# Autodesk Inventor assembly: Frame
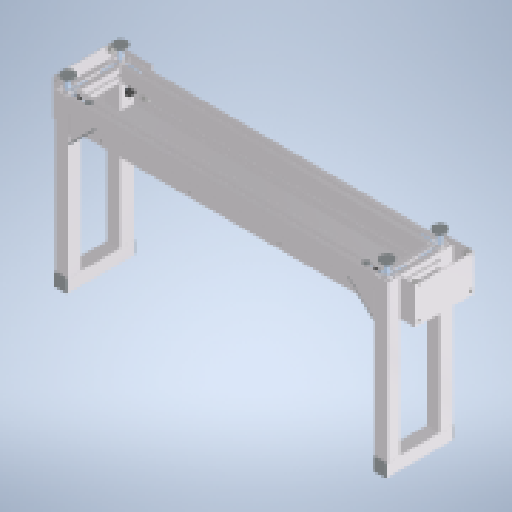
[picture p0: Inventor's stored thumbnail of the model, 512x512]
Saved by Autodesk Inventor 2025 (Build 290162010, 162A)
## iProperties
Created: 2025-01-18
Part Number: Frame
Document SubType Name: Assembly
Designer: Admin
Author: Admin
## Documents named in this file (34)
- C:\Users\Admin\GIT\HDVKBM\CAD\Krandemonstrator\Frame.iam
- C:\Users\Admin\GIT\HDVKBM\CAD\Krandemonstrator\item_61193_profil-x-8-40x40-2no180-_930_high\item_61193_profil-x-8-40x40-2no180-_930_high.ipt
- C:\Users\Admin\GIT\HDVKBM\CAD\Krandemonstrator\item_49291_profil-x-8-40x40-leicht-_120_high\item_49291_profil-x-8-40x40-leicht-_120_high.ipt
- C:\Users\Admin\GIT\HDVKBM\CAD\Krandemonstrator\item_49288_profil-x-8-40x40-4no-lei_200_high\item_49288_profil-x-8-40x40-4no-lei_200_high.ipt
- C:\Users\Admin\GIT\HDVKBM\CAD\Krandemonstrator\item_49288_profil-x-8-40x40-4no-lei_475_high\item_49288_profil-x-8-40x40-4no-lei_475_high.ipt
- C:\Users\Admin\GIT\HDVKBM\CAD\Krandemonstrator\item_67284_automatik-verbindungssat__high\item_67284_automatik-verbindungssat__high.ipt
- C:\Users\Admin\GIT\HDVKBM\CAD\Krandemonstrator\item_63697_stellfuss-d40-m8x60-grau_35_0_high\item_63697_stellfuss-d40-m8x60-grau_35_0_high.ipt
- C:\Users\Admin\GIT\HDVKBM\CAD\Krandemonstrator\item_62716_abdeckkappe-8-40x40-grau__high\item_62716_abdeckkappe-8-40x40-grau__high.ipt
- C:\Users\Admin\GIT\HDVKBM\CAD\Krandemonstrator\item_48996_automatik-verbindungssat__high\item_48996_automatik-verbindungssat__high.ipt
- C:\Users\Admin\GIT\HDVKBM\CAD\Krandemonstrator\item_41123_winkel-8-80x80-zn-weissa__high\item_41123_winkel-8-80x80-zn-weissa__high.ipt
- C:\Users\Admin\GIT\HDVKBM\CAD\Krandemonstrator\item_2618_nutenstein-8-st-m8-verzi__high\item_2618_nutenstein-8-st-m8-verzi__high.ipt
- C:\Users\Admin\Documents\Inventor\Content Center Files\R2025\de-DE\AS 1420\AS 1420 - 1973 - M8 x 16.ipt
- C:\Users\Admin\GIT\HDVKBM\CAD\Krandemonstrator\item_62758_winkel-abdeckkappe-8-80x__high\item_62758_winkel-abdeckkappe-8-80x__high.ipt
- C:\Users\Admin\GIT\HDVKBM\CAD\Krandemonstrator\item_43452_stellfuss-d30-m6x45-schw_20_0_high\item_43452_stellfuss-d30-m6x45-schw_20_0_high.ipt
- C:\Users\Admin\GIT\HDVKBM\CAD\Krandemonstrator\item_2623_nutenstein-8-st-m6-verzi__high\item_2623_nutenstein-8-st-m6-verzi__high.ipt
- C:\Users\Admin\GIT\HDVKBM\CAD\Krandemonstrator\item_42005_nutenstein-8-st-m5-verzi__high\item_42005_nutenstein-8-st-m5-verzi__high.ipt
- C:\Users\Admin\GIT\HDVKBM\CAD\Krandemonstrator\item_67777_winkel-5-20-weissalumini__high\item_67777_winkel-5-20-weissalumini__high.ipt
- C:\Users\Admin\GIT\HDVKBM\CAD\Krandemonstrator\item_68092_befestigungssatz-5-2-4mm_2_high\item_68092_befestigungssatz-5-2-4mm_2_high.ipt
- C:\Users\Admin\Documents\Inventor\Content Center Files\R2025\de-DE\DIN 7991(2)\DIN 7991 - M5x12.ipt
- C:\Users\Admin\GIT\HDVKBM\CAD\Krandemonstrator\item_47308_blech-al-2mm-naturfarben_1100_180_high\item_47308_blech-al-2mm-naturfarben_1100_180_high.ipt
- C:\Users\Admin\Documents\Inventor\Content Center Files\R2025\de-DE\DIN 7991(2)\DIN 7991 - M5x16.ipt
- C:\Users\Admin\Documents\Inventor\Content Center Files\R2025\de-DE\DIN 7991(2)\DIN 7991 - M4x8.ipt
- C:\Users\Admin\GIT\HDVKBM\CAD\Krandemonstrator\item_37006_nutenstein-5-st-m4-verzi__high\item_37006_nutenstein-5-st-m4-verzi__high.ipt
- C:\Users\Admin\GIT\HDVKBM\CAD\Krandemonstrator\item_47308_blech-al-2mm-naturfarben_110_1100_high\item_47308_blech-al-2mm-naturfarben_110_1100_high.ipt
- C:\Users\Admin\GIT\HDVKBM\CAD\Krandemonstrator\item_37003_profil-5-20x20-natur-370_1096_high\item_37003_profil-5-20x20-natur-370_1096_high.ipt
- C:\Users\Admin\GIT\HDVKBM\CAD\Krandemonstrator\item_43774_profil-5-20x20-1n-natur-_1096_high\item_43774_profil-5-20x20-1n-natur-_1096_high.ipt
- C:\Users\Admin\GIT\HDVKBM\CAD\Krandemonstrator\item_47308_blech-al-2mm-naturfarben_178_110_high\item_47308_blech-al-2mm-naturfarben_178_110_high.ipt
- C:\Users\Admin\GIT\HDVKBM\CAD\Krandemonstrator\item_47308_blech-al-2mm-naturfarben_120_90_high\item_47308_blech-al-2mm-naturfarben_120_90_high.ipt
- C:\Users\Admin\Documents\Inventor\Content Center Files\R2025\de-DE\DIN 7991(1)\DIN 7991 - M5  x  10.ipt
- C:\Users\Admin\GIT\HDVKBM\CAD\Krandemonstrator\Frameblock.ipt
- C:\Users\Admin\GIT\HDVKBM\CAD\Krandemonstrator\item_47308_blech-al-2mm-naturfarben_120_90_high\item_47308_blech-al-2mm-naturfarben_120_90_highLH.ipt
- C:\Users\Admin\Documents\Inventor\Content Center Files\R2025\de-DE\DIN 7991(2)\DIN 7991 - M3x8.ipt
- C:\Users\Admin\Documents\Inventor\Content Center Files\R2025\de-DE\DIN 7991(2)\DIN 7991 - M4x20.ipt
- C:\Users\Admin\Documents\Inventor\Content Center Files\R2025\de-DE\DIN 7991(1)\DIN 7991 - M4  x  8.ipt
## Components (126 placed, 33 different names)
1. Frameblock:1 — Starr:73, Starr:84, Passend:24
2. Frameblock:2 — Starr:74, Starr:83, Passend:23
3. Frameblock:3 — Starr:75
4. Frameblock:4 — Starr:76, Passend:16, Starr:82
5. Frameblock:5 — Starr:78
6. Frameblock:6 — Starr:77, Starr:81, Passend:11
7. Frameblock:7 — Starr:79
8. Frameblock:8 — Starr:80
9. DIN 7991 M3x8:1 — Passend:9
10. DIN 7991 M3x8:2 — Passend:10
11. item_37006_nutenstein-5-st-m4-verzi__high:5 — Starr:81
12. item_37006_nutenstein-5-st-m4-verzi__high:6 — Starr:84
13. DIN 7991 M4x20:1 — Passend:11
14. DIN 7991 M3x8:3 — Passend:12
15. DIN 7991 M3x8:4 — Passend:13
16. DIN 7991 M3x8:5 — Passend:14
17. DIN 7991 M3x8:6 — Passend:15
18. DIN 7991 M4x20:2 — Passend:16
19. item_37006_nutenstein-5-st-m4-verzi__high:7 — Starr:82
20. item_37006_nutenstein-5-st-m4-verzi__high:8 — Starr:83
21. DIN 7991 M3x8:7 — Passend:17
22. DIN 7991 M3x8:8 — Passend:18
23. DIN 7991 M3x8:9 — Passend:19
24. DIN 7991 M3x8:10 — Passend:20
25. DIN 7991 M3x8:11 — Passend:21
26. DIN 7991 M3x8:12 — Passend:22
27. DIN 7991 M4x20:3 — Passend:23
28. DIN 7991 M4x20:4 — Passend:24
29. DIN 7991 - ersetzt durch DIN EN ISO 10642 M4  x  8:1 — Starr:85, Starr:91
30. DIN 7991 - ersetzt durch DIN EN ISO 10642 M4  x  8:2 — Starr:86, Starr:92
31. DIN 7991 - ersetzt durch DIN EN ISO 10642 M4  x  8:3 — Starr:87, Starr:89
32. DIN 7991 - ersetzt durch DIN EN ISO 10642 M4  x  8:4 — Starr:88, Starr:90
33. item_37006_nutenstein-5-st-m4-verzi__high:9 — Starr:91
34. item_37006_nutenstein-5-st-m4-verzi__high:10 — Starr:92
35. item_37006_nutenstein-5-st-m4-verzi__high:11 — Starr:90
36. item_37006_nutenstein-5-st-m4-verzi__high:12 — Starr:89
37. item_61193_profil-x-8-40x40-2no180-_930_high:1 — Starr:12, Starr:13, Starr:14
38. item_61193_profil-x-8-40x40-2no180-_930_high:2 — Starr:17, Starr:27, Planar:1, Planar:2, Starr:47, Starr:48, Planar:68, Verschiebbar:70
39. item_49291_profil-x-8-40x40-leicht-_120_high:1 — Starr:7, Starr:8, Starr:9
40. item_49291_profil-x-8-40x40-leicht-_120_high:2 — Starr:24, Starr:25, Starr:26
41. item_49288_profil-x-8-40x40-4no-lei_200_high:1 — Starr:18, Starr:19, Starr:21, Starr:23
42. item_49288_profil-x-8-40x40-4no-lei_200_high:2 — Starr:2, Starr:4, Starr:5, Starr:6
43. item_49288_profil-x-8-40x40-4no-lei_475_high:1 — Starr:20, Starr:21, Starr:28, Starr:41, Verschiebbar:6
44. item_49288_profil-x-8-40x40-4no-lei_475_high:2 — Starr:22, Starr:23, Starr:25, Starr:27, Starr:29, Verschiebbar:2, Verschiebbar:4
45. item_49288_profil-x-8-40x40-4no-lei_475_high:3 — Starr:3, Starr:4, Starr:11, Starr:17, Verschiebbar:1, Verschiebbar:3, Planar:71
46. item_49288_profil-x-8-40x40-4no-lei_475_high:4 — Starr:1, Starr:2, Starr:9, Starr:10, Starr:14, Starr:43, Verschiebbar:5
47. item_67284_automatik-verbindungssat__high:1 — Starr:1
48. item_67284_automatik-verbindungssat__high:2 — Starr:20
49. item_67284_automatik-verbindungssat__high:3 — Starr:3
50. item_67284_automatik-verbindungssat__high:11 — Starr:22
51. item_67284_automatik-verbindungssat__high:4 — Starr:24
52. item_67284_automatik-verbindungssat__high:12 — Starr:26
53. item_67284_automatik-verbindungssat__high:5 — Starr:12
54. item_67284_automatik-verbindungssat__high:6 — Starr:13
55. item_67284_automatik-verbindungssat__high:7 — Starr:8
56. item_67284_automatik-verbindungssat__high:8 — Starr:7
57. item_48996_automatik-verbindungssat__high:1 — Starr:47
58. item_48996_automatik-verbindungssat__high:2 — Starr:48
59. item_63697_stellfuss-d40-m8x60-grau_35_0_high:1 — Starr:10
60. item_63697_stellfuss-d40-m8x60-grau_35_0_high:2 — Starr:11
61. item_63697_stellfuss-d40-m8x60-grau_35_0_high:3 — Starr:28
62. item_63697_stellfuss-d40-m8x60-grau_35_0_high:4 — Starr:29
63. item_62716_abdeckkappe-8-40x40-grau__high:1 — Starr:5
64. item_62716_abdeckkappe-8-40x40-grau__high:2 — Starr:6
65. item_62716_abdeckkappe-8-40x40-grau__high:3 — Starr:18
66. item_62716_abdeckkappe-8-40x40-grau__high:4 — Starr:19
67. item_41123_winkel-8-80x80-zn-weissa__high:1 — Einfügen:3, Einfügen:4, Einfügen:7, Einfügen:8, Verschiebbar:2, Planar:2, Starr:38
68. item_41123_winkel-8-80x80-zn-weissa__high:2 — Einfügen:1, Einfügen:2, Einfügen:5, Einfügen:6, Verschiebbar:1, Planar:1, Starr:39
69. item_2618_nutenstein-8-st-m8-verzi__high:5 — Starr:37
70. item_2618_nutenstein-8-st-m8-verzi__high:3 — Starr:36
71. item_2618_nutenstein-8-st-m8-verzi__high:2 — Starr:31
72. item_2618_nutenstein-8-st-m8-verzi__high:6 — Starr:30
73. item_2618_nutenstein-8-st-m8-verzi__high:4 — Starr:32
74. item_2618_nutenstein-8-st-m8-verzi__high:8 — Starr:33
75. item_2618_nutenstein-8-st-m8-verzi__high:1 — Starr:34
76. item_2618_nutenstein-8-st-m8-verzi__high:7 — Starr:35
77. AS 1420 - Metrisch M8 x 16:1 — Einfügen:1, Starr:37
78. AS 1420 - Metrisch M8 x 16:2 — Einfügen:2, Starr:36
79. AS 1420 - Metrisch M8 x 16:3 — Einfügen:3, Starr:35
80. AS 1420 - Metrisch M8 x 16:4 — Einfügen:4, Starr:34
81. AS 1420 - Metrisch M8 x 16:5 — Einfügen:5, Starr:31
82. AS 1420 - Metrisch M8 x 16:6 — Einfügen:6, Starr:30
83. AS 1420 - Metrisch M8 x 16:7 — Einfügen:7, Starr:33
84. AS 1420 - Metrisch M8 x 16:8 — Einfügen:8, Starr:32
85. item_62758_winkel-abdeckkappe-8-80x__high:1 — Starr:38
86. item_62758_winkel-abdeckkappe-8-80x__high:2 — Starr:39
87. item_2623_nutenstein-8-st-m6-verzi__high:2 — Starr:42, Starr:43
88. item_2623_nutenstein-8-st-m6-verzi__high:1 — Starr:40, Starr:41
89. item_43452_stellfuss-d30-m6x45-schw_20_0_high:1 — Starr:40
90. item_43452_stellfuss-d30-m6x45-schw_20_0_high:2 — Starr:42
91. DIN 7991 - ersetzt durch DIN EN ISO 10642 M5  x  10:2 — Passend:5
92. DIN 7991 - ersetzt durch DIN EN ISO 10642 M5  x  10:1 — Passend:6
93. DIN 7991 - ersetzt durch DIN EN ISO 10642 M5  x  10:3 — Passend:7
94. DIN 7991 - ersetzt durch DIN EN ISO 10642 M5  x  10:4 — Passend:8
95. item_47308_blech-al-2mm-naturfarben_110_1100_high:1 — Starr:64, Starr:65, Starr:66, Starr:67, Planar:71, Starr:68, Verschiebbar:70, Starr:69, Starr:70, Passend:9, Passend:22
96. item_47308_blech-al-2mm-naturfarben_178_110_high:1 — Starr:69, Starr:71, Passend:5, Passend:6, Starr:80, Passend:20, Passend:21
97. item_47308_blech-al-2mm-naturfarben_178_110_high:2 — Starr:70, Starr:72, Passend:7, Passend:8, Starr:79, Passend:10, Passend:12
98. item_47308_blech-al-2mm-naturfarben_120_90_highLH:1 — Starr:72, Starr:76, Starr:77, Starr:78, Passend:13, Passend:14, Passend:15
99. item_47308_blech-al-2mm-naturfarben_120_90_high:2 — Starr:71, Starr:73, Starr:74, Starr:75, Passend:17, Passend:18, Passend:19
100. DIN 7991 M4x8:1 — Starr:60, Starr:67
101. DIN 7991 M4x8:2 — Starr:62, Starr:64
102. DIN 7991 M4x8:3 — Starr:61, Starr:66
103. DIN 7991 M4x8:4 — Starr:63, Starr:65
104. item_43774_profil-5-20x20-1n-natur-_1096_high:1 — Planar:73, Planar:76
105. item_37006_nutenstein-5-st-m4-verzi__high:1 — Starr:61
106. item_37006_nutenstein-5-st-m4-verzi__high:2 — Starr:63
107. item_37006_nutenstein-5-st-m4-verzi__high:3 — Starr:62
108. item_37006_nutenstein-5-st-m4-verzi__high:4 — Starr:60
109. item_47308_blech-al-2mm-naturfarben_1100_180_high:1 — Planar:68, Starr:68, Planar:76, Starr:85, Starr:86, Starr:87, Starr:88
110. item_37003_profil-5-20x20-natur-370_1096_high:1
111. DIN 7991 M5x12:1 — Passend:1
112. DIN 7991 M5x12:2 — Passend:2
113. DIN 7991 M5x16:2 — Passend:3
114. DIN 7991 M5x16:1 — Passend:4
115. item_42005_nutenstein-8-st-m5-verzi__high:1 — Starr:45
116. item_42005_nutenstein-8-st-m5-verzi__high:2 — Starr:44
117. item_42005_nutenstein-8-st-m5-verzi__high:3 — Starr:52
118. item_42005_nutenstein-8-st-m5-verzi__high:4 — Starr:53
119. item_67777_winkel-5-20-weissalumini__high:1 — Starr:44, Starr:49, Passend:1, Verschiebbar:6, Planar:73
120. item_67777_winkel-5-20-weissalumini__high:2 — Starr:45, Starr:46, Passend:2, Verschiebbar:5
121. item_67777_winkel-5-20-weissalumini__high:3 — Starr:50, Passend:3, Starr:53, Verschiebbar:4
122. item_67777_winkel-5-20-weissalumini__high:4 — Starr:51, Passend:4, Starr:52, Verschiebbar:3
123. item_68092_befestigungssatz-5-2-4mm_2_high:1 — Starr:49
124. item_68092_befestigungssatz-5-2-4mm_2_high:2 — Starr:46
125. item_68092_befestigungssatz-5-2-4mm_2_high:3 — Starr:50
126. item_68092_befestigungssatz-5-2-4mm_2_high:4 — Starr:51
## Relationships (138: WeldJoint 84, Mate 24, PlanarJoint 14, Insert 8, TranslationJoint 8)
- Starr:1 [WeldJoint]: item_49288_profil-x-8-40x40-4no-lei_475_high:4 ↔ item_67284_automatik-verbindungssat__high:1
- Starr:2 [WeldJoint]: item_49288_profil-x-8-40x40-4no-lei_200_high:2 ↔ item_49288_profil-x-8-40x40-4no-lei_475_high:4
- Starr:3 [WeldJoint]: item_49288_profil-x-8-40x40-4no-lei_475_high:3 ↔ item_67284_automatik-verbindungssat__high:3
- Starr:4 [WeldJoint]: item_49288_profil-x-8-40x40-4no-lei_200_high:2 ↔ item_49288_profil-x-8-40x40-4no-lei_475_high:3
- Starr:5 [WeldJoint]: item_49288_profil-x-8-40x40-4no-lei_200_high:2 ↔ item_62716_abdeckkappe-8-40x40-grau__high:1
- Starr:6 [WeldJoint]: item_49288_profil-x-8-40x40-4no-lei_200_high:2 ↔ item_62716_abdeckkappe-8-40x40-grau__high:2
- Starr:7 [WeldJoint]: item_49291_profil-x-8-40x40-leicht-_120_high:1 ↔ item_67284_automatik-verbindungssat__high:8
- Starr:8 [WeldJoint]: item_49291_profil-x-8-40x40-leicht-_120_high:1 ↔ item_67284_automatik-verbindungssat__high:7
- Starr:9 [WeldJoint]: item_49291_profil-x-8-40x40-leicht-_120_high:1 ↔ item_49288_profil-x-8-40x40-4no-lei_475_high:4
- Starr:10 [WeldJoint]: item_49288_profil-x-8-40x40-4no-lei_475_high:4 ↔ item_63697_stellfuss-d40-m8x60-grau_35_0_high:1
- Starr:11 [WeldJoint]: item_49288_profil-x-8-40x40-4no-lei_475_high:3 ↔ item_63697_stellfuss-d40-m8x60-grau_35_0_high:2
- Starr:12 [WeldJoint]: item_61193_profil-x-8-40x40-2no180-_930_high:1 ↔ item_67284_automatik-verbindungssat__high:5
- Starr:13 [WeldJoint]: item_61193_profil-x-8-40x40-2no180-_930_high:1 ↔ item_67284_automatik-verbindungssat__high:6
- Starr:14 [WeldJoint]: item_61193_profil-x-8-40x40-2no180-_930_high:1 ↔ item_49288_profil-x-8-40x40-4no-lei_475_high:4
- Starr:17 [WeldJoint]: item_61193_profil-x-8-40x40-2no180-_930_high:2 ↔ item_49288_profil-x-8-40x40-4no-lei_475_high:3
- Starr:18 [WeldJoint]: item_49288_profil-x-8-40x40-4no-lei_200_high:1 ↔ item_62716_abdeckkappe-8-40x40-grau__high:3
- Starr:19 [WeldJoint]: item_49288_profil-x-8-40x40-4no-lei_200_high:1 ↔ item_62716_abdeckkappe-8-40x40-grau__high:4
- Starr:20 [WeldJoint]: item_49288_profil-x-8-40x40-4no-lei_475_high:1 ↔ item_67284_automatik-verbindungssat__high:2
- Starr:21 [WeldJoint]: item_49288_profil-x-8-40x40-4no-lei_200_high:1 ↔ item_49288_profil-x-8-40x40-4no-lei_475_high:1
- Starr:22 [WeldJoint]: item_49288_profil-x-8-40x40-4no-lei_475_high:2 ↔ item_67284_automatik-verbindungssat__high:11
- Starr:23 [WeldJoint]: item_49288_profil-x-8-40x40-4no-lei_200_high:1 ↔ item_49288_profil-x-8-40x40-4no-lei_475_high:2
- Starr:24 [WeldJoint]: item_49291_profil-x-8-40x40-leicht-_120_high:2 ↔ item_67284_automatik-verbindungssat__high:4
- Starr:25 [WeldJoint]: item_49291_profil-x-8-40x40-leicht-_120_high:2 ↔ item_49288_profil-x-8-40x40-4no-lei_475_high:2
- Starr:26 [WeldJoint]: item_49291_profil-x-8-40x40-leicht-_120_high:2 ↔ item_67284_automatik-verbindungssat__high:12
- Starr:27 [WeldJoint]: item_61193_profil-x-8-40x40-2no180-_930_high:2 ↔ item_49288_profil-x-8-40x40-4no-lei_475_high:2
- Starr:28 [WeldJoint]: item_49288_profil-x-8-40x40-4no-lei_475_high:1 ↔ item_63697_stellfuss-d40-m8x60-grau_35_0_high:3
- Starr:29 [WeldJoint]: item_49288_profil-x-8-40x40-4no-lei_475_high:2 ↔ item_63697_stellfuss-d40-m8x60-grau_35_0_high:4
- Einfügen:1 [Insert]: item_41123_winkel-8-80x80-zn-weissa__high:2 ↔ AS 1420 - Metrisch M8 x 16:1
- Einfügen:2 [Insert]: item_41123_winkel-8-80x80-zn-weissa__high:2 ↔ AS 1420 - Metrisch M8 x 16:2
- Einfügen:3 [Insert]: item_41123_winkel-8-80x80-zn-weissa__high:1 ↔ AS 1420 - Metrisch M8 x 16:3
- Einfügen:4 [Insert]: item_41123_winkel-8-80x80-zn-weissa__high:1 ↔ AS 1420 - Metrisch M8 x 16:4
- Einfügen:5 [Insert]: item_41123_winkel-8-80x80-zn-weissa__high:2 ↔ AS 1420 - Metrisch M8 x 16:5
- Einfügen:6 [Insert]: item_41123_winkel-8-80x80-zn-weissa__high:2 ↔ AS 1420 - Metrisch M8 x 16:6
- Einfügen:7 [Insert]: item_41123_winkel-8-80x80-zn-weissa__high:1 ↔ AS 1420 - Metrisch M8 x 16:7
- Einfügen:8 [Insert]: item_41123_winkel-8-80x80-zn-weissa__high:1 ↔ AS 1420 - Metrisch M8 x 16:8
- Starr:30 [WeldJoint]: item_2618_nutenstein-8-st-m8-verzi__high:6 ↔ AS 1420 - Metrisch M8 x 16:6
- Starr:31 [WeldJoint]: item_2618_nutenstein-8-st-m8-verzi__high:2 ↔ AS 1420 - Metrisch M8 x 16:5
- Starr:32 [WeldJoint]: item_2618_nutenstein-8-st-m8-verzi__high:4 ↔ AS 1420 - Metrisch M8 x 16:8
- Starr:33 [WeldJoint]: item_2618_nutenstein-8-st-m8-verzi__high:8 ↔ AS 1420 - Metrisch M8 x 16:7
- Starr:34 [WeldJoint]: item_2618_nutenstein-8-st-m8-verzi__high:1 ↔ AS 1420 - Metrisch M8 x 16:4
- Starr:35 [WeldJoint]: item_2618_nutenstein-8-st-m8-verzi__high:7 ↔ AS 1420 - Metrisch M8 x 16:3
- Starr:36 [WeldJoint]: item_2618_nutenstein-8-st-m8-verzi__high:3 ↔ AS 1420 - Metrisch M8 x 16:2
- Starr:37 [WeldJoint]: item_2618_nutenstein-8-st-m8-verzi__high:5 ↔ AS 1420 - Metrisch M8 x 16:1
- Verschiebbar:1 [TranslationJoint]: item_49288_profil-x-8-40x40-4no-lei_475_high:3 ↔ item_41123_winkel-8-80x80-zn-weissa__high:2
- Planar:1: item_61193_profil-x-8-40x40-2no180-_930_high:2 ↔ item_41123_winkel-8-80x80-zn-weissa__high:2
- Verschiebbar:2 [TranslationJoint]: item_49288_profil-x-8-40x40-4no-lei_475_high:2 ↔ item_41123_winkel-8-80x80-zn-weissa__high:1
- Planar:2: item_61193_profil-x-8-40x40-2no180-_930_high:2 ↔ item_41123_winkel-8-80x80-zn-weissa__high:1
- Starr:38 [WeldJoint]: item_41123_winkel-8-80x80-zn-weissa__high:1 ↔ item_62758_winkel-abdeckkappe-8-80x__high:1
- Starr:39 [WeldJoint]: item_41123_winkel-8-80x80-zn-weissa__high:2 ↔ item_62758_winkel-abdeckkappe-8-80x__high:2
- Starr:40 [WeldJoint]: item_2623_nutenstein-8-st-m6-verzi__high:1 ↔ item_43452_stellfuss-d30-m6x45-schw_20_0_high:1
- Starr:41 [WeldJoint] (-60 mm): item_49288_profil-x-8-40x40-4no-lei_475_high:1 ↔ item_2623_nutenstein-8-st-m6-verzi__high:1
- Starr:42 [WeldJoint]: item_2623_nutenstein-8-st-m6-verzi__high:2 ↔ item_43452_stellfuss-d30-m6x45-schw_20_0_high:2
- Starr:43 [WeldJoint] (-60 mm): item_49288_profil-x-8-40x40-4no-lei_475_high:4 ↔ item_2623_nutenstein-8-st-m6-verzi__high:2
- Starr:44 [WeldJoint] (-5 mm): item_42005_nutenstein-8-st-m5-verzi__high:2 ↔ item_67777_winkel-5-20-weissalumini__high:1
- Starr:45 [WeldJoint] (-5 mm): item_42005_nutenstein-8-st-m5-verzi__high:1 ↔ item_67777_winkel-5-20-weissalumini__high:2
- Starr:46 [WeldJoint]: item_67777_winkel-5-20-weissalumini__high:2 ↔ item_68092_befestigungssatz-5-2-4mm_2_high:2
- Starr:47 [WeldJoint]: item_61193_profil-x-8-40x40-2no180-_930_high:2 ↔ item_48996_automatik-verbindungssat__high:1
- Starr:48 [WeldJoint]: item_61193_profil-x-8-40x40-2no180-_930_high:2 ↔ item_48996_automatik-verbindungssat__high:2
- Starr:49 [WeldJoint]: item_67777_winkel-5-20-weissalumini__high:1 ↔ item_68092_befestigungssatz-5-2-4mm_2_high:1
- Passend:1 [Mate]: DIN 7991 M5x12:1 ↔ item_67777_winkel-5-20-weissalumini__high:1
- Passend:2 [Mate]: DIN 7991 M5x12:2 ↔ item_67777_winkel-5-20-weissalumini__high:2
- Starr:50 [WeldJoint]: item_67777_winkel-5-20-weissalumini__high:3 ↔ item_68092_befestigungssatz-5-2-4mm_2_high:3
- Starr:51 [WeldJoint]: item_67777_winkel-5-20-weissalumini__high:4 ↔ item_68092_befestigungssatz-5-2-4mm_2_high:4
- Passend:3 [Mate]: DIN 7991 M5x16:2 ↔ item_67777_winkel-5-20-weissalumini__high:3
- Passend:4 [Mate]: DIN 7991 M5x16:1 ↔ item_67777_winkel-5-20-weissalumini__high:4
- Starr:52 [WeldJoint] (-5 mm): item_42005_nutenstein-8-st-m5-verzi__high:3 ↔ item_67777_winkel-5-20-weissalumini__high:4
- Starr:53 [WeldJoint] (-5 mm): item_42005_nutenstein-8-st-m5-verzi__high:4 ↔ item_67777_winkel-5-20-weissalumini__high:3
- Verschiebbar:3 [TranslationJoint] (2 mm): item_49288_profil-x-8-40x40-4no-lei_475_high:3 ↔ item_67777_winkel-5-20-weissalumini__high:4
- Verschiebbar:4 [TranslationJoint]: item_49288_profil-x-8-40x40-4no-lei_475_high:2 ↔ item_67777_winkel-5-20-weissalumini__high:3
- [PlanarJoint]: item_37003_profil-5-20x20-natur-370_1096_high:1 ↔ item_67777_winkel-5-20-weissalumini__high:4
- [PlanarJoint]: item_37003_profil-5-20x20-natur-370_1096_high:1 ↔ item_67777_winkel-5-20-weissalumini__high:3
- Verschiebbar:5 [TranslationJoint]: item_49288_profil-x-8-40x40-4no-lei_475_high:4 ↔ item_67777_winkel-5-20-weissalumini__high:2
- Verschiebbar:6 [TranslationJoint]: item_49288_profil-x-8-40x40-4no-lei_475_high:1 ↔ item_67777_winkel-5-20-weissalumini__high:1
- [PlanarJoint]: item_47308_blech-al-2mm-naturfarben_1100_180_high:1 ↔ item_37003_profil-5-20x20-natur-370_1096_high:1
- Starr:60 [WeldJoint]: DIN 7991 M4x8:1 ↔ item_37006_nutenstein-5-st-m4-verzi__high:4
- Starr:61 [WeldJoint]: DIN 7991 M4x8:3 ↔ item_37006_nutenstein-5-st-m4-verzi__high:1
- Starr:62 [WeldJoint]: DIN 7991 M4x8:2 ↔ item_37006_nutenstein-5-st-m4-verzi__high:3
- Starr:63 [WeldJoint]: DIN 7991 M4x8:4 ↔ item_37006_nutenstein-5-st-m4-verzi__high:2
- Planar:68 (75 mm): item_61193_profil-x-8-40x40-2no180-_930_high:2 ↔ item_47308_blech-al-2mm-naturfarben_1100_180_high:1
- Starr:64 [WeldJoint]: item_47308_blech-al-2mm-naturfarben_110_1100_high:1 ↔ DIN 7991 M4x8:2
- Starr:65 [WeldJoint]: item_47308_blech-al-2mm-naturfarben_110_1100_high:1 ↔ DIN 7991 M4x8:4
- Starr:66 [WeldJoint]: item_47308_blech-al-2mm-naturfarben_110_1100_high:1 ↔ DIN 7991 M4x8:3
- Starr:67 [WeldJoint]: item_47308_blech-al-2mm-naturfarben_110_1100_high:1 ↔ DIN 7991 M4x8:1
- [PlanarJoint]: item_47308_blech-al-2mm-naturfarben_110_1100_high:1 ↔ item_37003_profil-5-20x20-natur-370_1096_high:1
- [PlanarJoint]: item_47308_blech-al-2mm-naturfarben_110_1100_high:1 ↔ item_37003_profil-5-20x20-natur-370_1096_high:1
- [TranslationJoint]: item_47308_blech-al-2mm-naturfarben_110_1100_high:1 ↔ item_37003_profil-5-20x20-natur-370_1096_high:1
- Planar:71: item_49288_profil-x-8-40x40-4no-lei_475_high:3 ↔ item_47308_blech-al-2mm-naturfarben_110_1100_high:1
- Starr:68 [WeldJoint]: item_47308_blech-al-2mm-naturfarben_110_1100_high:1 ↔ item_47308_blech-al-2mm-naturfarben_1100_180_high:1
- Verschiebbar:70 [TranslationJoint]: item_61193_profil-x-8-40x40-2no180-_930_high:2 ↔ item_47308_blech-al-2mm-naturfarben_110_1100_high:1
- [PlanarJoint]: item_43774_profil-5-20x20-1n-natur-_1096_high:1 ↔ item_47308_blech-al-2mm-naturfarben_1100_180_high:1
- Planar:73: item_43774_profil-5-20x20-1n-natur-_1096_high:1 ↔ item_67777_winkel-5-20-weissalumini__high:1
- [PlanarJoint]: item_43774_profil-5-20x20-1n-natur-_1096_high:1 ↔ item_67777_winkel-5-20-weissalumini__high:2
- [PlanarJoint]: item_49288_profil-x-8-40x40-4no-lei_475_high:4 ↔ item_43774_profil-5-20x20-1n-natur-_1096_high:1
- Planar:76 (-2 mm): item_43774_profil-5-20x20-1n-natur-_1096_high:1 ↔ item_47308_blech-al-2mm-naturfarben_1100_180_high:1
- Starr:69 [WeldJoint]: item_47308_blech-al-2mm-naturfarben_110_1100_high:1 ↔ item_47308_blech-al-2mm-naturfarben_178_110_high:1
- Starr:70 [WeldJoint]: item_47308_blech-al-2mm-naturfarben_110_1100_high:1 ↔ item_47308_blech-al-2mm-naturfarben_178_110_high:2
- Starr:71 [WeldJoint]: item_47308_blech-al-2mm-naturfarben_178_110_high:1 ↔ item_47308_blech-al-2mm-naturfarben_120_90_high:2
- Starr:72 [WeldJoint]: item_47308_blech-al-2mm-naturfarben_178_110_high:2 ↔ item_47308_blech-al-2mm-naturfarben_120_90_highLH:1
- Passend:5 [Mate]: DIN 7991 - ersetzt durch DIN EN ISO 10642 M5  x  10:2 ↔ item_47308_blech-al-2mm-naturfarben_178_110_high:1
- Passend:6 [Mate]: DIN 7991 - ersetzt durch DIN EN ISO 10642 M5  x  10:1 ↔ item_47308_blech-al-2mm-naturfarben_178_110_high:1
- Passend:7 [Mate]: DIN 7991 - ersetzt durch DIN EN ISO 10642 M5  x  10:3 ↔ item_47308_blech-al-2mm-naturfarben_178_110_high:2
- Passend:8 [Mate]: DIN 7991 - ersetzt durch DIN EN ISO 10642 M5  x  10:4 ↔ item_47308_blech-al-2mm-naturfarben_178_110_high:2
- Starr:73 [WeldJoint]: Frameblock:1 ↔ item_47308_blech-al-2mm-naturfarben_120_90_high:2
- Starr:74 [WeldJoint]: Frameblock:2 ↔ item_47308_blech-al-2mm-naturfarben_120_90_high:2
- Starr:75 [WeldJoint]: Frameblock:3 ↔ item_47308_blech-al-2mm-naturfarben_120_90_high:2
- Starr:76 [WeldJoint]: Frameblock:4 ↔ item_47308_blech-al-2mm-naturfarben_120_90_highLH:1
- Starr:77 [WeldJoint]: Frameblock:6 ↔ item_47308_blech-al-2mm-naturfarben_120_90_highLH:1
- Starr:78 [WeldJoint]: Frameblock:5 ↔ item_47308_blech-al-2mm-naturfarben_120_90_highLH:1
- Starr:79 [WeldJoint]: Frameblock:7 ↔ item_47308_blech-al-2mm-naturfarben_178_110_high:2
- Starr:80 [WeldJoint]: Frameblock:8 ↔ item_47308_blech-al-2mm-naturfarben_178_110_high:1
- Passend:9 [Mate]: DIN 7991 M3x8:1 ↔ item_47308_blech-al-2mm-naturfarben_110_1100_high:1
- Passend:10 [Mate]: DIN 7991 M3x8:2 ↔ item_47308_blech-al-2mm-naturfarben_178_110_high:2
- Starr:81 [WeldJoint]: Frameblock:6 ↔ item_37006_nutenstein-5-st-m4-verzi__high:5
- Passend:11 [Mate]: Frameblock:6 ↔ DIN 7991 M4x20:1
- Passend:12 [Mate]: DIN 7991 M3x8:3 ↔ item_47308_blech-al-2mm-naturfarben_178_110_high:2
- Passend:13 [Mate]: DIN 7991 M3x8:4 ↔ item_47308_blech-al-2mm-naturfarben_120_90_highLH:1
- Passend:14 [Mate]: DIN 7991 M3x8:5 ↔ item_47308_blech-al-2mm-naturfarben_120_90_highLH:1
- Passend:15 [Mate]: DIN 7991 M3x8:6 ↔ item_47308_blech-al-2mm-naturfarben_120_90_highLH:1
- Passend:16 [Mate]: Frameblock:4 ↔ DIN 7991 M4x20:2
- Starr:82 [WeldJoint]: Frameblock:4 ↔ item_37006_nutenstein-5-st-m4-verzi__high:7
- Passend:17 [Mate]: DIN 7991 M3x8:7 ↔ item_47308_blech-al-2mm-naturfarben_120_90_high:2
- Passend:18 [Mate]: DIN 7991 M3x8:8 ↔ item_47308_blech-al-2mm-naturfarben_120_90_high:2
- Passend:19 [Mate]: DIN 7991 M3x8:9 ↔ item_47308_blech-al-2mm-naturfarben_120_90_high:2
- Passend:20 [Mate]: DIN 7991 M3x8:10 ↔ item_47308_blech-al-2mm-naturfarben_178_110_high:1
- Passend:21 [Mate]: DIN 7991 M3x8:11 ↔ item_47308_blech-al-2mm-naturfarben_178_110_high:1
- Passend:22 [Mate]: DIN 7991 M3x8:12 ↔ item_47308_blech-al-2mm-naturfarben_110_1100_high:1
- Starr:83 [WeldJoint]: Frameblock:2 ↔ item_37006_nutenstein-5-st-m4-verzi__high:8
- Passend:23 [Mate]: Frameblock:2 ↔ DIN 7991 M4x20:3
- Starr:84 [WeldJoint]: Frameblock:1 ↔ item_37006_nutenstein-5-st-m4-verzi__high:6
- Passend:24 [Mate]: Frameblock:1 ↔ DIN 7991 M4x20:4
- Starr:85 [WeldJoint]: DIN 7991 - ersetzt durch DIN EN ISO 10642 M4  x  8:1 ↔ item_47308_blech-al-2mm-naturfarben_1100_180_high:1
- Starr:86 [WeldJoint]: DIN 7991 - ersetzt durch DIN EN ISO 10642 M4  x  8:2 ↔ item_47308_blech-al-2mm-naturfarben_1100_180_high:1
- Starr:87 [WeldJoint]: DIN 7991 - ersetzt durch DIN EN ISO 10642 M4  x  8:3 ↔ item_47308_blech-al-2mm-naturfarben_1100_180_high:1
- Starr:88 [WeldJoint]: DIN 7991 - ersetzt durch DIN EN ISO 10642 M4  x  8:4 ↔ item_47308_blech-al-2mm-naturfarben_1100_180_high:1
- Starr:89 [WeldJoint]: DIN 7991 - ersetzt durch DIN EN ISO 10642 M4  x  8:3 ↔ item_37006_nutenstein-5-st-m4-verzi__high:12
- Starr:90 [WeldJoint]: DIN 7991 - ersetzt durch DIN EN ISO 10642 M4  x  8:4 ↔ item_37006_nutenstein-5-st-m4-verzi__high:11
- Starr:91 [WeldJoint]: DIN 7991 - ersetzt durch DIN EN ISO 10642 M4  x  8:1 ↔ item_37006_nutenstein-5-st-m4-verzi__high:9
- Starr:92 [WeldJoint]: DIN 7991 - ersetzt durch DIN EN ISO 10642 M4  x  8:2 ↔ item_37006_nutenstein-5-st-m4-verzi__high:10
